# Autodesk Inventor assembly: stainless steel engine
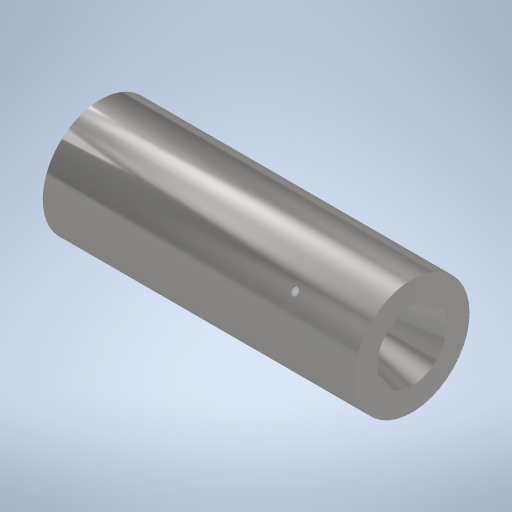
[picture p0: Inventor's stored thumbnail of the model, 512x512]
Saved by Autodesk Inventor 2023 (Build 270158000, 158)
## iProperties
Created: 2022-09-19
Part Number: stainless steel engine
Document SubType Name: Assembly
Designer: station
Author: station
## Documents named in this file (6)
- C:\Users\station\Documents\Project\Liquid-engine-cooling-system\design files\ethanol engine 6\stainless steel engine.iam
- C:\Users\station\Documents\Project\Liquid-engine-cooling-system\design files\ethanol engine 6\stainless steel final chamber.ipt
- C:\Users\station\Documents\Project\Liquid-engine-cooling-system\design files\ethanol engine 6\stainless steel final nozzle.ipt
- C:\Users\station\Documents\Project\Liquid-engine-cooling-system\design files\ethanol engine 6\stainless steel space.ipt
- C:\Users\station\Documents\Project\Liquid-engine-cooling-system\design files\ethanol engine 6\stainless steel outer wall.ipt
- C:\Users\station\Documents\Project\Liquid-engine-cooling-system\design files\ethanol engine 6\stainless steel end.ipt
## Components (5 placed, 5 different names)
1. stainless steel final chamber:1 — Mate:1, Mate:2
2. stainless steel final nozzle:1 — Mate:1, Mate:2, Mate:3, Mate:4, Mate:5, Flush:1
3. stainless steel space:1 — Mate:3, Mate:4
4. stainless steel outer wall:1 — Mate:5, Flush:1, Mate:6, Mate:7
5. stainless steel end:1 — Mate:6, Mate:7
## Relationships (8: Mate 7, Flush 1)
- Mate:1: stainless steel final chamber:1 ↔ stainless steel final nozzle:1
- Mate:2: stainless steel final chamber:1 ↔ stainless steel final nozzle:1
- Mate:3: stainless steel final nozzle:1 ↔ stainless steel space:1
- Mate:4 (13.716 mm): stainless steel final nozzle:1 ↔ stainless steel space:1
- Mate:5: stainless steel final nozzle:1 ↔ stainless steel outer wall:1
- Flush:1: stainless steel final nozzle:1 ↔ stainless steel outer wall:1
- Mate:6: stainless steel outer wall:1 ↔ stainless steel end:1
- Mate:7: stainless steel outer wall:1 ↔ stainless steel end:1
